# Autodesk Inventor assembly: Pushfit-Adapter_MIR
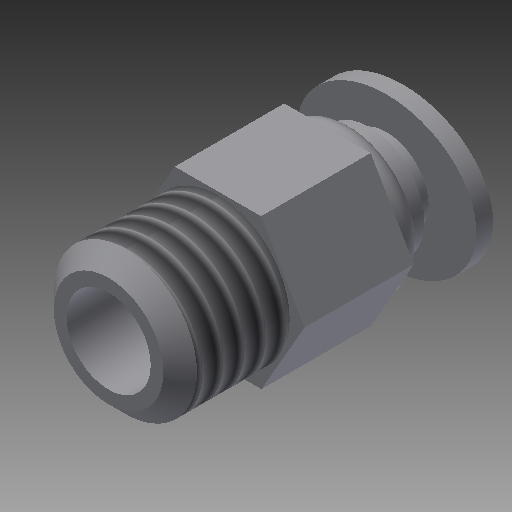
[picture p0: Inventor's stored thumbnail of the model, 512x512]
Saved by Autodesk Inventor 2017 (Build 210142000, 142)
## iProperties
Created: 2016-07-07
Part Number: Pushfit-Adapter_MIR
Document SubType Name: Assembly
Designer: User
Author: joshmamo
## Documents named in this file (3)
- C:\All INVENTOR\SL-Inventor\SL-Beast 3D Printer\Pushfit-Adapter_MIR.iam
- C:\All INVENTOR\SL-Inventor\SL-Beast 3D Printer\Pushfit-Adapter_MIR.ipt
- C:\All INVENTOR\SL-Inventor\SL-Beast 3D Printer\Pushfit-adapter-cap_MIR.ipt
## Components (2 placed, 2 different names)
1. Pushfit-Adapter_MIR:1 — Flush:1
2. Pushfit-adapter-cap_MIR:1 — Flush:1
## Relationships (1: Mate 1)
- Flush:1 [Mate]: Pushfit-Adapter_MIR:1 ↔ Pushfit-adapter-cap_MIR:1
